# Autodesk Inventor assembly: 276-2162
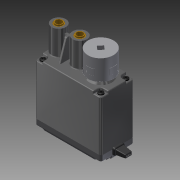
[picture p0: Inventor's stored thumbnail of the model, 180x180]
Saved by Autodesk Inventor 2013 (Build 170138000, 138)
## iProperties
Category: Sensors
Company: Autodesk Inc.
Created: 2012-04-11
Part Number: 276-2162
Document SubType Name: Assembly
Designer: Autodesk Inc.
Catalog Web Link: http://www.vexrobotics.com/276-2162.html
Vendor: VEX
Author: Autodesk Inc.
## Documents named in this file (9)
- C:\Data Folder\VEX 2012\VEX KOP Uploads\2013\Metric\Sensors\3 Wire Servo.iam
- C:\Data Folder\VEX 2012\VEX KOP Uploads\2013\Metric\Sensors\Components\Insert-Nut-632-Simple.ipt
- C:\Data Folder\VEX 2012\VEX KOP Uploads\2013\Metric\Sensors\Components\Vex-Motor-Top-Housing.ipt
- C:\Data Folder\VEX 2012\VEX KOP Uploads\2013\Metric\Sensors\Components\Vex-Motor-Output-Gear.ipt
- C:\Data Folder\VEX 2012\VEX KOP Uploads\2013\Metric\Sensors\Components\Vex-Motor-Bottom-Plate.ipt
- C:\Data Folder\VEX 2012\VEX KOP Uploads\2013\Metric\Sensors\Components\Vex-Motor-Bottom-Housing.ipt
- C:\Data Folder\VEX 2012\VEX KOP Uploads\2013\Metric\Sensors\Components\Vex-Wire-Support.ipt
- C:\Data Folder\VEX 2012\VEX KOP Uploads\2013\Metric\Sensors\Components\Motor-Clutch.ipt
- C:\Data Folder\VEX 2012\VEX KOP Uploads\2013\Metric\Sensors\Components\Cross Recessed Binding Head Machine Screw - Type I - Inch 0 - 80 - 3_16.ipt
## Components (16 placed, 8 different names)
1. Insert-Nut-632-Simple:1 — Flush:1, Mate:1
2. Vex-Motor-Top-Housing:1 — Flush:1, Flush:2, Mate:1, Mate:2, Flush:3, Mate:3, Mate:5, Mate:6, Flush:4, Flush:5, Mate:7, Insert:1, Insert:2, Insert:3, Insert:4, Mate:8
3. Vex-Motor-Output-Gear:1 — Flush:3, Mate:4, Mate:8
4. Insert-Nut-632-Simple:2 — Flush:2, Mate:2
5. Vex-Motor-Bottom-Plate:1 — Insert:5, Insert:6, Insert:7, Insert:8, Mate:9, Mate:10, Mate:11
6. Vex-Motor-Bottom-Housing:1 — Mate:5, Mate:6, Flush:4, Flush:5, Mate:7, Mate:9, Mate:10, Mate:11
7. Vex-Wire-Support:1
8. Motor-Clutch:1 — Mate:3, Mate:4
9. Cross Recessed Binding Head Machine Screw - Type I - Inch 0 - 80 - 3_16:1 — Insert:1
10. Cross Recessed Binding Head Machine Screw - Type I - Inch 0 - 80 - 3_16:2 — Insert:2
11. Cross Recessed Binding Head Machine Screw - Type I - Inch 0 - 80 - 3_16:3 — Insert:3
12. Cross Recessed Binding Head Machine Screw - Type I - Inch 0 - 80 - 3_16:4 — Insert:4
13. Cross Recessed Binding Head Machine Screw - Type I - Inch 0 - 80 - 3_16:5 — Insert:7
14. Cross Recessed Binding Head Machine Screw - Type I - Inch 0 - 80 - 3_16:6 — Insert:8
15. Cross Recessed Binding Head Machine Screw - Type I - Inch 0 - 80 - 3_16:7 — Insert:6
16. Cross Recessed Binding Head Machine Screw - Type I - Inch 0 - 80 - 3_16:8 — Insert:5
## Relationships (24: Mate 11, Insert 8, Flush 5)
- Flush:1 (-0.6858 mm): Insert-Nut-632-Simple:1 ↔ Vex-Motor-Top-Housing:1
- Flush:2 (-0.6858 mm): Vex-Motor-Top-Housing:1 ↔ Insert-Nut-632-Simple:2
- Mate:1: Insert-Nut-632-Simple:1 ↔ Vex-Motor-Top-Housing:1
- Mate:2: Vex-Motor-Top-Housing:1 ↔ Insert-Nut-632-Simple:2
- Flush:3: Vex-Motor-Top-Housing:1 ↔ Vex-Motor-Output-Gear:1
- Mate:3: Vex-Motor-Top-Housing:1 ↔ Motor-Clutch:1
- Mate:4: Vex-Motor-Output-Gear:1 ↔ Motor-Clutch:1
- Mate:5: Vex-Motor-Top-Housing:1 ↔ Vex-Motor-Bottom-Housing:1
- Mate:6: Vex-Motor-Top-Housing:1 ↔ Vex-Motor-Bottom-Housing:1
- Flush:4: Vex-Motor-Top-Housing:1 ↔ Vex-Motor-Bottom-Housing:1
- Flush:5: Vex-Motor-Top-Housing:1 ↔ Vex-Motor-Bottom-Housing:1
- Mate:7: Vex-Motor-Top-Housing:1 ↔ Vex-Motor-Bottom-Housing:1
- Insert:1: Vex-Motor-Top-Housing:1 ↔ Cross Recessed Binding Head Machine Screw - Type I - Inch 0 - 80 - 3_16:1
- Insert:2: Vex-Motor-Top-Housing:1 ↔ Cross Recessed Binding Head Machine Screw - Type I - Inch 0 - 80 - 3_16:2
- Insert:3: Vex-Motor-Top-Housing:1 ↔ Cross Recessed Binding Head Machine Screw - Type I - Inch 0 - 80 - 3_16:3
- Insert:4: Vex-Motor-Top-Housing:1 ↔ Cross Recessed Binding Head Machine Screw - Type I - Inch 0 - 80 - 3_16:4
- Insert:5: Vex-Motor-Bottom-Plate:1 ↔ Cross Recessed Binding Head Machine Screw - Type I - Inch 0 - 80 - 3_16:8
- Insert:6: Vex-Motor-Bottom-Plate:1 ↔ Cross Recessed Binding Head Machine Screw - Type I - Inch 0 - 80 - 3_16:7
- Insert:7: Vex-Motor-Bottom-Plate:1 ↔ Cross Recessed Binding Head Machine Screw - Type I - Inch 0 - 80 - 3_16:5
- Insert:8: Vex-Motor-Bottom-Plate:1 ↔ Cross Recessed Binding Head Machine Screw - Type I - Inch 0 - 80 - 3_16:6
- Mate:8: Vex-Motor-Top-Housing:1 ↔ Vex-Motor-Output-Gear:1
- Mate:9: Vex-Motor-Bottom-Plate:1 ↔ Vex-Motor-Bottom-Housing:1
- Mate:10: Vex-Motor-Bottom-Plate:1 ↔ Vex-Motor-Bottom-Housing:1
- Mate:11: Vex-Motor-Bottom-Plate:1 ↔ Vex-Motor-Bottom-Housing:1
